# Autodesk Inventor assembly: Housing
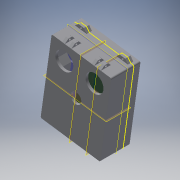
[picture p0: Inventor's stored thumbnail of the model, 180x180]
Saved by Autodesk Inventor 2017 (Build 210142000, 142)
## iProperties
Created: 2017-05-28
Part Number: Housing
Document SubType Name: Assembly
Designer: William
Author: William
## Documents named in this file (5)
- F:\Dropbox\University\METR4901\Australia\Housing Design\Design 2\Housing.iam
- F:\Dropbox\University\METR4901\Australia\Housing Design\Design 2\Base.ipt
- F:\Dropbox\University\METR4901\Australia\Housing Design\Design 2\PCB Holder.ipt
- F:\Dropbox\University\METR4901\Australia\Housing Design\Design 2\Top.ipt
- F:\Dropbox\University\METR4901\Australia\Housing Design\Design 2\SensorPlatformV3.iam
## Components (4 placed, 4 different names)
1. Base:1 — Mate:1, Mate:2, Mate:3, Mate:4, Mate:5, Mate:9
2. PCB Holder:1 — Mate:1, Mate:2, Mate:3, Mate:6, Mate:7, Mate:8
3. Top:1 — Mate:4, Mate:5, Mate:9
4. SensorPlatformV3:1 [sub-assembly] — Mate:6, Mate:7, Mate:8
## Relationships (9: Mate 9)
- Mate:1: Base:1 ↔ PCB Holder:1
- Mate:2: Base:1 ↔ PCB Holder:1
- Mate:3: Base:1 ↔ PCB Holder:1
- Mate:4: Base:1 ↔ Top:1
- Mate:5: Base:1 ↔ Top:1
- Mate:6: PCB Holder:1 ↔ SensorPlatformV3:1
- Mate:7: PCB Holder:1 ↔ SensorPlatformV3:1
- Mate:8: PCB Holder:1 ↔ SensorPlatformV3:1
- Mate:9: Base:1 ↔ Top:1
